# Autodesk Inventor assembly: Trunk
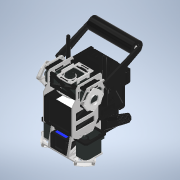
[picture p0: Inventor's stored thumbnail of the model, 180x180]
Saved by Autodesk Inventor 2020.4 (Build 244396000, 396)
## iProperties
Created: 2021-09-10
Part Number: Trunk
Document SubType Name: Assembly
Designer: Masato
Mass: 1534.62 g
Surface Area: 5672.23 cm^2
Volume: 933.606 cm^3
Density: 1.64375 g/cm^3
Author: Masato
## Documents named in this file (25)
- C:\Users\Masato\Documents\Inventor\CIT Brains_Inventor\OpenPlatform_ver3_0\UpperBody\Trunk\Trunk.iam
- C:\Users\Masato\Documents\Inventor\CIT Brains_Inventor\OpenPlatform_ver3_0\UpperBody\Trunk\Trunk_horizontal_frame_01.ipt
- C:\Users\Masato\Documents\Inventor\CIT Brains_Inventor\OpenPlatform_ver3_0\UpperBody\Trunk\Trunk_horizontal_frame_02.ipt
- C:\Users\Masato\Documents\Inventor\CIT Brains_Inventor\OpenPlatform_ver3_0\UpperBody\Trunk\Trunk_horizontal_frame_03.ipt
- C:\Users\Masato\Documents\Inventor\CIT Brains_Inventor\OpenPlatform_ver3_0\UpperBody\Trunk\Trunk_horizontal_frame_04.ipt
- C:\Users\Masato\Documents\Inventor\CIT Brains_Inventor\OpenPlatform_ver3_0\UpperBody\Trunk\Trunk_horizontal_frame_05.ipt
- C:\Users\Masato\Documents\Inventor\CIT Brains_Inventor\OpenPlatform_ver3_0\UpperBody\Trunk\Trunk_vertical_frame_02.ipt
- C:\Users\Masato\Documents\Inventor\CIT Brains_Inventor\OpenPlatform_ver3_0\UpperBody\Trunk\Trunk_vertical_frame_03.ipt
- C:\Users\Masato\Documents\Inventor\CIT Brains_Inventor\OpenPlatform_ver3_0\UpperBody\Trunk\Trunk_vertical_frame_04.ipt
- C:\Users\Masato\Documents\Inventor\CIT Brains_Inventor\OpenPlatform_ver3_0\UpperBody\Trunk\Trunk_vertical_frame_05.ipt
- C:\Users\Masato\Documents\Inventor\CIT Brains_Inventor\OpenPlatform_ver3_0\UpperBody\Trunk\Trunk_vertical_frame_06.ipt
- C:\Users\Masato\Documents\Inventor\CIT Brains_Inventor\OpenPlatform_ver3_0\Ready_Made\B3M11xx.ipt
- C:\Users\Masato\Documents\Inventor\CIT Brains_Inventor\OpenPlatform_ver3_0\Ready_Made\S3-07-3W.ipt
- C:\Users\Masato\Documents\Inventor\CIT Brains_Inventor\OpenPlatform_ver3_0\Ready_Made\ASU-375H.ipt
- C:\Users\Masato\Documents\Inventor\CIT Brains_Inventor\OpenPlatform_ver3_0\UpperBody\Trunk\RearBumper.ipt
- C:\Users\Masato\Documents\Inventor\CIT Brains_Inventor\OpenPlatform_ver3_0\UpperBody\Trunk\RearBumper_MIR.ipt
- C:\Users\Masato\Documents\Inventor\CIT Brains_Inventor\OpenPlatform_ver3_0\Ready_Made\MSU-306-03.ipt
- C:\Users\Masato\Documents\Inventor\CIT Brains_Inventor\OpenPlatform_ver3_0\Ready_Made\SLSBF7-130-M3-N3.ipt
- C:\Users\Masato\Documents\Inventor\CIT Brains_Inventor\OpenPlatform_ver3_0\Ready_Made\B3M10xx.ipt
- C:\Users\Masato\Documents\Inventor\CIT Brains_Inventor\OpenPlatform_ver3_0\Ready_Made\SGB-100.ipt
- C:\Users\Masato\Documents\Inventor\CIT Brains_Inventor\OpenPlatform_ver3_0\UpperBody\Cockpit\Cockpit.iam
- C:\Users\Masato\Documents\Inventor\CIT Brains_Inventor\OpenPlatform_ver3_0\UpperBody\Trunk\Trunk_vertical_frame_04_MIR.ipt
- C:\Users\Masato\Documents\Inventor\CIT Brains_Inventor\OpenPlatform_ver3_0\UpperBody\Trunk\Trunk_vertical_frame_01.ipt
- C:\Users\Masato\Documents\Inventor\CIT Brains_Inventor\OpenPlatform_ver3_0\UpperBody\Trunk\Trunk_vertical_frame_01_MIR.ipt
- C:\Users\Masato\Documents\Inventor\CIT Brains_Inventor\OpenPlatform_ver3_0\下半身\付け根ロール\付け根ロール_サブフレーム_1_3.ipt
## Components (69 placed, 24 different names)
1. Trunk_horizontal_frame_01:1 — メイト:1, フラッシュ:14, 挿入:1, 挿入:2, 挿入:3, 挿入:4, 挿入:5, 挿入:6, 挿入:7, 挿入:8, 挿入:93, 挿入:94, 挿入:95, 挿入:96, 挿入:97, 挿入:98, 挿入:100, 角度:23, 挿入:196, 挿入:197, 挿入:198, 挿入:199, 挿入:211
2. Trunk_horizontal_frame_02:1 — 挿入:9, 挿入:10, 挿入:11, 挿入:12
3. Trunk_horizontal_frame_03:1 — 挿入:172, 挿入:173, 挿入:174, 挿入:175, 挿入:176, 挿入:177, 挿入:178, 挿入:179
4. Trunk_horizontal_frame_03:2 — 挿入:180, 挿入:181, 挿入:182, 挿入:183, 挿入:184, 挿入:185, 挿入:186, 挿入:187
5. Trunk_horizontal_frame_04:1 — 挿入:115, 挿入:116, 挿入:117, 挿入:118, 挿入:172, 挿入:173, 挿入:181, 挿入:182
6. Trunk_horizontal_frame_04:2 — 挿入:154, 挿入:155, 挿入:156, 挿入:157, 挿入:174, 挿入:175, 挿入:185, 挿入:187
7. Trunk_horizontal_frame_05:1 — 挿入:111, 挿入:112, 挿入:126, 挿入:127
8. Trunk_horizontal_frame_05:2 — 挿入:162, 挿入:163, 挿入:164, 挿入:165
9. Trunk_horizontal_frame_05:3 — 挿入:107, 挿入:108, 挿入:138, 挿入:139
10. Trunk_horizontal_frame_05:4 — 挿入:166, 挿入:167, 挿入:168, 挿入:169
11. Trunk_vertical_frame_01:1 — 挿入:196, 挿入:197, 角度:35, 角度:36, 挿入:200, 挿入:201, 挿入:206, 挿入:207
12. Trunk_vertical_frame_01_MIR:1 — 挿入:198, 挿入:199, 角度:37, 角度:38, 挿入:202, 挿入:203, 挿入:204, 挿入:205, メイト:23, メイト:24, メイト:25
13. Trunk_vertical_frame_02:1 — フラッシュ:16, メイト:17, フラッシュ:18, フラッシュ:20, フラッシュ:21, メイト:22
14. Trunk_vertical_frame_02:2 — フラッシュ:16, メイト:17, フラッシュ:18, メイト:19
15. Trunk_vertical_frame_02:3 — フラッシュ:15, メイト:18, フラッシュ:17, フラッシュ:19, フラッシュ:20, フラッシュ:21, メイト:21, メイト:20
16. Trunk_vertical_frame_02:4 — フラッシュ:15, メイト:18, フラッシュ:17, メイト:25
17. Trunk_vertical_frame_03:1 — 挿入:101, 挿入:102, 挿入:103, 挿入:111, 挿入:112, 挿入:115, 挿入:116, 挿入:156, 挿入:157, 挿入:164, 挿入:165, フラッシュ:19, メイト:21, 挿入:208
18. Trunk_vertical_frame_03:2 — 挿入:104, 挿入:105, 挿入:106, 挿入:107, 挿入:108, 挿入:117, 挿入:118, 挿入:154, 挿入:155, 挿入:168, 挿入:169, メイト:22
19. Trunk_vertical_frame_04:1 — 挿入:138, 挿入:139, 挿入:142, 挿入:143, 挿入:144, 挿入:145, 挿入:146, 挿入:147, 挿入:148, 挿入:149, 角度:31, 角度:32, 挿入:150, 挿入:151, 挿入:166, 挿入:167
20. Trunk_vertical_frame_04_MIR:1 — 挿入:124, 挿入:125, 挿入:126, 挿入:127, 挿入:128, 挿入:129, 挿入:132, 挿入:133, 挿入:134, 挿入:135, 挿入:136, 挿入:137, 角度:33, 角度:34, 挿入:152, 挿入:153, 挿入:162, 挿入:163
21. Trunk_vertical_frame_05:1 — 角度:17, 角度:18, 挿入:75, 挿入:76, 角度:21, 挿入:79, メイト:16
22. Trunk_vertical_frame_05:2 — 角度:19, 挿入:77, 挿入:78, 角度:20, 角度:22, 挿入:80
23. Trunk_vertical_frame_06:1 — 挿入:192, 挿入:193, 挿入:194, 挿入:195
24. Trunk_vertical_frame_06:2 — 挿入:188, 挿入:189, 挿入:190, 挿入:191
25. 付け根ロール_サブフレーム_1_3:1 — 挿入:209, 挿入:215, 挿入:216, 挿入:217
26. 付け根ロール_サブフレーム_1_3:2 — 挿入:210, 挿入:212, 挿入:213, 挿入:214
27. 付け根ロール_サブフレーム_1_3:3 — 挿入:221, 挿入:222, 挿入:223, 挿入:224
28. 付け根ロール_サブフレーム_1_3:4 — 挿入:218, 挿入:219, 挿入:220, 挿入:225
29. RearBumper:1 — 挿入:204, 挿入:205
30. RearBumper_MIR:1 — 挿入:206, 挿入:207
31. B3M11xx:1 — 挿入:1, 挿入:2, 挿入:3, 挿入:4, 挿入:11, 挿入:12, 角度:39
32. B3M11xx:2 — 挿入:5, 挿入:6, 挿入:7, 挿入:8, 挿入:9, 挿入:10
33. B3M11xx:3 — 挿入:176, 挿入:177, 挿入:178, 挿入:179, 挿入:180, 挿入:183, 挿入:184, 挿入:186
34. B3M10xx:4 — 挿入:124, 挿入:125, 挿入:128, 挿入:129, 挿入:188, 挿入:189, 挿入:190, 挿入:191
35. B3M10xx:5 — 挿入:142, 挿入:143, 挿入:144, 挿入:145, 挿入:192, 挿入:193, 挿入:194, 挿入:195
36. S3-07-3W:1 — 角度:37, 挿入:202
37. S3-07-3W:2 — 角度:38, 挿入:203
38. S3-07-3W:3 — 角度:36, 挿入:201
39. S3-07-3W:4 — 角度:35, 挿入:200
40. S3-07-3W:5 — 角度:33, 挿入:152
41. S3-07-3W:6 — 角度:34, 挿入:153
42. S3-07-3W:7 — 角度:31, 挿入:150
43. S3-07-3W:8 — 角度:32, 挿入:151
44. ASU-375H:1 — フラッシュ:9, フラッシュ:10, フラッシュ:11, フラッシュ:12, 挿入:101, 挿入:104, メイト:19, メイト:20, メイト:23, メイト:24
45. ASU-375H:2 — フラッシュ:9, フラッシュ:11, 挿入:102, 挿入:105
46. ASU-375H:3 — フラッシュ:10, フラッシュ:12, 挿入:103, 挿入:106
47. MSU-306-03:1 — 角度:12, 挿入:133, 挿入:222
48. MSU-306-03:2 — 角度:10, 角度:11, 角度:12, 挿入:132, 挿入:221
49. MSU-306-03:3 — 角度:11, 挿入:135, 挿入:224
50. MSU-306-03:4 — 角度:10, 挿入:134, 挿入:223
51. MSU-306-03:5 — 角度:17, 挿入:75, 挿入:136
52. MSU-306-03:6 — 角度:18, 挿入:76, 挿入:137
53. MSU-306-03:7 — 角度:14, 角度:15, 角度:16, 挿入:146, 挿入:218
54. MSU-306-03:8 — 角度:14, 挿入:147, 挿入:220
55. MSU-306-03:9 — 角度:15, 挿入:149, 挿入:225
56. MSU-306-03:10 — 角度:16, 挿入:148, 挿入:219
57. MSU-306-03:11 — 角度:19, 挿入:77
58. MSU-306-03:12 — 挿入:78, 角度:20
59. SLSBF7-130-M3-N3:1 — 角度:21, 角度:22, 挿入:79, 挿入:80, メイト:15
60. SGB-100:1 — メイト:15, メイト:16
61. MSU-306-03:13 — 挿入:93, 角度:23, 角度:24, 角度:25, 角度:26, 角度:27, 角度:28, 角度:29, 角度:30, 挿入:217
62. MSU-306-03:14 — 挿入:95, 角度:25, 挿入:209
63. MSU-306-03:15 — 挿入:94, 角度:24, 挿入:216
64. MSU-306-03:16 — 挿入:96, 角度:26, 挿入:215
65. MSU-306-03:17 — 挿入:97, 角度:27, 挿入:210
66. MSU-306-03:18 — 挿入:98, 角度:30, 挿入:214
67. MSU-306-03:19 — 角度:28, 挿入:211, 挿入:212
68. MSU-306-03:20 — 挿入:100, 角度:29, 挿入:213
69. Cockpit:1 [sub-assembly] — 挿入:208, 角度:39
## Relationships (184: Insert 131, Angle 29, Mate 12, Flush 12)
- メイト:1 [Mate]: Trunk_horizontal_frame_01:1
- フラッシュ:14 [Flush]: Trunk_horizontal_frame_01:1
- 挿入:1 [Insert]: Trunk_horizontal_frame_01:1 ↔ B3M11xx:1
- 挿入:2 [Insert]: Trunk_horizontal_frame_01:1 ↔ B3M11xx:1
- 挿入:3 [Insert]: Trunk_horizontal_frame_01:1 ↔ B3M11xx:1
- 挿入:4 [Insert]: Trunk_horizontal_frame_01:1 ↔ B3M11xx:1
- 挿入:5 [Insert]: Trunk_horizontal_frame_01:1 ↔ B3M11xx:2
- 挿入:6 [Insert]: Trunk_horizontal_frame_01:1 ↔ B3M11xx:2
- 挿入:7 [Insert]: Trunk_horizontal_frame_01:1 ↔ B3M11xx:2
- 挿入:8 [Insert]: Trunk_horizontal_frame_01:1 ↔ B3M11xx:2
- 挿入:9 [Insert]: Trunk_horizontal_frame_02:1 ↔ B3M11xx:2
- 挿入:10 [Insert]: Trunk_horizontal_frame_02:1 ↔ B3M11xx:2
- 挿入:11 [Insert]: Trunk_horizontal_frame_02:1 ↔ B3M11xx:1
- 挿入:12 [Insert]: Trunk_horizontal_frame_02:1 ↔ B3M11xx:1
- フラッシュ:9 [Flush]: ASU-375H:1 ↔ ASU-375H:2
- フラッシュ:10 [Flush]: ASU-375H:1 ↔ ASU-375H:3
- フラッシュ:11 [Flush]: ASU-375H:1 ↔ ASU-375H:2
- フラッシュ:12 [Flush]: ASU-375H:1 ↔ ASU-375H:3
- 角度:10 [Angle] (0 deg): MSU-306-03:2 ↔ MSU-306-03:4
- 角度:11 [Angle] (0 deg): MSU-306-03:2 ↔ MSU-306-03:3
- 角度:12 [Angle] (0 deg): MSU-306-03:1 ↔ MSU-306-03:2
- 角度:14 [Angle] (0 deg): MSU-306-03:7 ↔ MSU-306-03:8
- 角度:15 [Angle] (0 deg): MSU-306-03:7 ↔ MSU-306-03:9
- 角度:16 [Angle] (0 deg): MSU-306-03:7 ↔ MSU-306-03:10
- 角度:17 [Angle] (0 deg): Trunk_vertical_frame_05:1 ↔ MSU-306-03:5
- 角度:18 [Angle] (0 deg): Trunk_vertical_frame_05:1 ↔ MSU-306-03:6
- 挿入:75 [Insert]: Trunk_vertical_frame_05:1 ↔ MSU-306-03:5
- 挿入:76 [Insert]: Trunk_vertical_frame_05:1 ↔ MSU-306-03:6
- 角度:19 [Angle] (0 deg): Trunk_vertical_frame_05:2 ↔ MSU-306-03:11
- 挿入:77 [Insert]: Trunk_vertical_frame_05:2 ↔ MSU-306-03:11
- 挿入:78 [Insert]: Trunk_vertical_frame_05:2 ↔ MSU-306-03:12
- 角度:20 [Angle] (0 deg): Trunk_vertical_frame_05:2 ↔ MSU-306-03:12
- 角度:21 [Angle] (0 deg): Trunk_vertical_frame_05:1 ↔ SLSBF7-130-M3-N3:1
- 角度:22 [Angle] (0 deg): Trunk_vertical_frame_05:2 ↔ SLSBF7-130-M3-N3:1
- 挿入:79 [Insert]: Trunk_vertical_frame_05:1 ↔ SLSBF7-130-M3-N3:1
- 挿入:80 [Insert]: Trunk_vertical_frame_05:2 ↔ SLSBF7-130-M3-N3:1
- メイト:15 [Mate]: SLSBF7-130-M3-N3:1 ↔ SGB-100:1
- メイト:16 [Mate] (2.5 mm): Trunk_vertical_frame_05:1 ↔ SGB-100:1
- 挿入:93 [Insert]: Trunk_horizontal_frame_01:1 ↔ MSU-306-03:13
- 挿入:94 [Insert]: Trunk_horizontal_frame_01:1 ↔ MSU-306-03:15
- 挿入:95 [Insert]: Trunk_horizontal_frame_01:1 ↔ MSU-306-03:14
- 挿入:96 [Insert]: Trunk_horizontal_frame_01:1 ↔ MSU-306-03:16
- 挿入:97 [Insert]: Trunk_horizontal_frame_01:1 ↔ MSU-306-03:17
- 挿入:98 [Insert]: Trunk_horizontal_frame_01:1 ↔ MSU-306-03:18
- 挿入:100 [Insert]: Trunk_horizontal_frame_01:1 ↔ MSU-306-03:20
- 角度:23 [Angle] (0 deg): Trunk_horizontal_frame_01:1 ↔ MSU-306-03:13
- 角度:24 [Angle] (0 deg): MSU-306-03:13 ↔ MSU-306-03:15
- 角度:25 [Angle] (0 deg): MSU-306-03:13 ↔ MSU-306-03:14
- 角度:26 [Angle] (0 deg): MSU-306-03:13 ↔ MSU-306-03:16
- 角度:27 [Angle] (0 deg): MSU-306-03:13 ↔ MSU-306-03:17
- 角度:28 [Angle] (0 deg): MSU-306-03:13 ↔ MSU-306-03:19
- 角度:29 [Angle] (0 deg): MSU-306-03:13 ↔ MSU-306-03:20
- 角度:30 [Angle] (0 deg): MSU-306-03:13 ↔ MSU-306-03:18
- 挿入:101 [Insert]: Trunk_vertical_frame_03:1 ↔ ASU-375H:1
- 挿入:102 [Insert]: Trunk_vertical_frame_03:1 ↔ ASU-375H:2
- 挿入:103 [Insert]: Trunk_vertical_frame_03:1 ↔ ASU-375H:3
- 挿入:104 [Insert]: Trunk_vertical_frame_03:2 ↔ ASU-375H:1
- 挿入:105 [Insert]: Trunk_vertical_frame_03:2 ↔ ASU-375H:2
- 挿入:106 [Insert]: Trunk_vertical_frame_03:2 ↔ ASU-375H:3
- 挿入:107 [Insert]: Trunk_horizontal_frame_05:3 ↔ Trunk_vertical_frame_03:2
- 挿入:108 [Insert]: Trunk_horizontal_frame_05:3 ↔ Trunk_vertical_frame_03:2
- 挿入:111 [Insert]: Trunk_horizontal_frame_05:1 ↔ Trunk_vertical_frame_03:1
- 挿入:112 [Insert]: Trunk_horizontal_frame_05:1 ↔ Trunk_vertical_frame_03:1
- 挿入:115 [Insert]: Trunk_horizontal_frame_04:1 ↔ Trunk_vertical_frame_03:1
- 挿入:116 [Insert]: Trunk_horizontal_frame_04:1 ↔ Trunk_vertical_frame_03:1
- 挿入:117 [Insert]: Trunk_horizontal_frame_04:1 ↔ Trunk_vertical_frame_03:2
- 挿入:118 [Insert]: Trunk_horizontal_frame_04:1 ↔ Trunk_vertical_frame_03:2
- 挿入:124 [Insert]: Trunk_vertical_frame_04_MIR:1 ↔ B3M10xx:4
- 挿入:125 [Insert]: Trunk_vertical_frame_04_MIR:1 ↔ B3M10xx:4
- 挿入:126 [Insert]: Trunk_horizontal_frame_05:1 ↔ Trunk_vertical_frame_04_MIR:1
- 挿入:127 [Insert]: Trunk_horizontal_frame_05:1 ↔ Trunk_vertical_frame_04_MIR:1
- 挿入:128 [Insert]: Trunk_vertical_frame_04_MIR:1 ↔ B3M10xx:4
- 挿入:129 [Insert]: Trunk_vertical_frame_04_MIR:1 ↔ B3M10xx:4
- 挿入:132 [Insert]: Trunk_vertical_frame_04_MIR:1 ↔ MSU-306-03:2
- 挿入:133 [Insert]: Trunk_vertical_frame_04_MIR:1 ↔ MSU-306-03:1
- 挿入:134 [Insert]: Trunk_vertical_frame_04_MIR:1 ↔ MSU-306-03:4
- 挿入:135 [Insert]: Trunk_vertical_frame_04_MIR:1 ↔ MSU-306-03:3
- 挿入:136 [Insert]: Trunk_vertical_frame_04_MIR:1 ↔ MSU-306-03:5
- 挿入:137 [Insert]: Trunk_vertical_frame_04_MIR:1 ↔ MSU-306-03:6
- 挿入:138 [Insert]: Trunk_horizontal_frame_05:3 ↔ Trunk_vertical_frame_04:1
- 挿入:139 [Insert]: Trunk_horizontal_frame_05:3 ↔ Trunk_vertical_frame_04:1
- 挿入:142 [Insert]: Trunk_vertical_frame_04:1 ↔ B3M10xx:5
- 挿入:143 [Insert]: Trunk_vertical_frame_04:1 ↔ B3M10xx:5
- 挿入:144 [Insert]: Trunk_vertical_frame_04:1 ↔ B3M10xx:5
- 挿入:145 [Insert]: Trunk_vertical_frame_04:1 ↔ B3M10xx:5
- 挿入:146 [Insert]: Trunk_vertical_frame_04:1 ↔ MSU-306-03:7
- 挿入:147 [Insert]: Trunk_vertical_frame_04:1 ↔ MSU-306-03:8
- 挿入:148 [Insert]: Trunk_vertical_frame_04:1 ↔ MSU-306-03:10
- 挿入:149 [Insert]: Trunk_vertical_frame_04:1 ↔ MSU-306-03:9
- 角度:31 [Angle] (0 deg): Trunk_vertical_frame_04:1 ↔ S3-07-3W:7
- 角度:32 [Angle] (0 deg): Trunk_vertical_frame_04:1 ↔ S3-07-3W:8
- 挿入:150 [Insert]: Trunk_vertical_frame_04:1 ↔ S3-07-3W:7
- 挿入:151 [Insert]: Trunk_vertical_frame_04:1 ↔ S3-07-3W:8
- 角度:33 [Angle] (0 deg): Trunk_vertical_frame_04_MIR:1 ↔ S3-07-3W:5
- 角度:34 [Angle] (0 deg): Trunk_vertical_frame_04_MIR:1 ↔ S3-07-3W:6
- 挿入:152 [Insert]: Trunk_vertical_frame_04_MIR:1 ↔ S3-07-3W:5
- 挿入:153 [Insert]: Trunk_vertical_frame_04_MIR:1 ↔ S3-07-3W:6
- 挿入:154 [Insert]: Trunk_horizontal_frame_04:2 ↔ Trunk_vertical_frame_03:2
- 挿入:155 [Insert]: Trunk_horizontal_frame_04:2 ↔ Trunk_vertical_frame_03:2
- 挿入:156 [Insert]: Trunk_horizontal_frame_04:2 ↔ Trunk_vertical_frame_03:1
- 挿入:157 [Insert]: Trunk_horizontal_frame_04:2 ↔ Trunk_vertical_frame_03:1
- 挿入:162 [Insert]: Trunk_horizontal_frame_05:2 ↔ Trunk_vertical_frame_04_MIR:1
- 挿入:163 [Insert]: Trunk_horizontal_frame_05:2 ↔ Trunk_vertical_frame_04_MIR:1
- 挿入:164 [Insert]: Trunk_horizontal_frame_05:2 ↔ Trunk_vertical_frame_03:1
- 挿入:165 [Insert]: Trunk_horizontal_frame_05:2 ↔ Trunk_vertical_frame_03:1
- 挿入:166 [Insert]: Trunk_horizontal_frame_05:4 ↔ Trunk_vertical_frame_04:1
- 挿入:167 [Insert]: Trunk_horizontal_frame_05:4 ↔ Trunk_vertical_frame_04:1
- 挿入:168 [Insert]: Trunk_horizontal_frame_05:4 ↔ Trunk_vertical_frame_03:2
- 挿入:169 [Insert]: Trunk_horizontal_frame_05:4 ↔ Trunk_vertical_frame_03:2
- 挿入:172 [Insert]: Trunk_horizontal_frame_03:1 ↔ Trunk_horizontal_frame_04:1
- 挿入:173 [Insert]: Trunk_horizontal_frame_03:1 ↔ Trunk_horizontal_frame_04:1
- 挿入:174 [Insert]: Trunk_horizontal_frame_03:1 ↔ Trunk_horizontal_frame_04:2
- 挿入:175 [Insert]: Trunk_horizontal_frame_03:1 ↔ Trunk_horizontal_frame_04:2
- 挿入:176 [Insert]: Trunk_horizontal_frame_03:1 ↔ B3M11xx:3
- 挿入:177 [Insert]: Trunk_horizontal_frame_03:1 ↔ B3M11xx:3
- 挿入:178 [Insert]: Trunk_horizontal_frame_03:1 ↔ B3M11xx:3
- 挿入:179 [Insert]: Trunk_horizontal_frame_03:1 ↔ B3M11xx:3
- 挿入:180 [Insert]: Trunk_horizontal_frame_03:2 ↔ B3M11xx:3
- 挿入:181 [Insert]: Trunk_horizontal_frame_03:2 ↔ Trunk_horizontal_frame_04:1
- 挿入:182 [Insert]: Trunk_horizontal_frame_03:2 ↔ Trunk_horizontal_frame_04:1
- 挿入:183 [Insert]: Trunk_horizontal_frame_03:2 ↔ B3M11xx:3
- 挿入:184 [Insert]: Trunk_horizontal_frame_03:2 ↔ B3M11xx:3
- 挿入:185 [Insert]: Trunk_horizontal_frame_03:2 ↔ Trunk_horizontal_frame_04:2
- 挿入:186 [Insert]: Trunk_horizontal_frame_03:2 ↔ B3M11xx:3
- 挿入:187 [Insert]: Trunk_horizontal_frame_03:2 ↔ Trunk_horizontal_frame_04:2
- 挿入:188 [Insert]: Trunk_vertical_frame_06:2 ↔ B3M10xx:4
- 挿入:189 [Insert]: Trunk_vertical_frame_06:2 ↔ B3M10xx:4
- 挿入:190 [Insert]: Trunk_vertical_frame_06:2 ↔ B3M10xx:4
- 挿入:191 [Insert]: Trunk_vertical_frame_06:2 ↔ B3M10xx:4
- 挿入:192 [Insert]: Trunk_vertical_frame_06:1 ↔ B3M10xx:5
- 挿入:193 [Insert]: Trunk_vertical_frame_06:1 ↔ B3M10xx:5
- 挿入:194 [Insert]: Trunk_vertical_frame_06:1 ↔ B3M10xx:5
- 挿入:195 [Insert]: Trunk_vertical_frame_06:1 ↔ B3M10xx:5
- フラッシュ:15 [Flush]: Trunk_vertical_frame_02:3 ↔ Trunk_vertical_frame_02:4
- フラッシュ:16 [Flush]: Trunk_vertical_frame_02:1 ↔ Trunk_vertical_frame_02:2
- メイト:17 [Mate]: Trunk_vertical_frame_02:1 ↔ Trunk_vertical_frame_02:2
- メイト:18 [Mate]: Trunk_vertical_frame_02:3 ↔ Trunk_vertical_frame_02:4
- フラッシュ:17 [Flush]: Trunk_vertical_frame_02:3 ↔ Trunk_vertical_frame_02:4
- フラッシュ:18 [Flush]: Trunk_vertical_frame_02:1 ↔ Trunk_vertical_frame_02:2
- フラッシュ:19 [Flush]: Trunk_vertical_frame_02:3 ↔ Trunk_vertical_frame_03:1
- フラッシュ:20 [Flush]: Trunk_vertical_frame_02:1 ↔ Trunk_vertical_frame_02:3
- メイト:19 [Mate] (0.01 mm): Trunk_vertical_frame_02:2 ↔ ASU-375H:1
- メイト:20 [Mate] (0.01 mm): Trunk_vertical_frame_02:3 ↔ ASU-375H:1
- フラッシュ:21 [Flush]: Trunk_vertical_frame_02:1 ↔ Trunk_vertical_frame_02:3
- メイト:21 [Mate]: Trunk_vertical_frame_02:3 ↔ Trunk_vertical_frame_03:1
- メイト:22 [Mate]: Trunk_vertical_frame_02:1 ↔ Trunk_vertical_frame_03:2
- 挿入:196 [Insert]: Trunk_horizontal_frame_01:1 ↔ Trunk_vertical_frame_01:1
- 挿入:197 [Insert]: Trunk_horizontal_frame_01:1 ↔ Trunk_vertical_frame_01:1
- 挿入:198 [Insert]: Trunk_horizontal_frame_01:1 ↔ Trunk_vertical_frame_01_MIR:1
- 挿入:199 [Insert]: Trunk_horizontal_frame_01:1 ↔ Trunk_vertical_frame_01_MIR:1
- 角度:35 [Angle] (0 deg): Trunk_vertical_frame_01:1 ↔ S3-07-3W:4
- 角度:36 [Angle] (0 deg): Trunk_vertical_frame_01:1 ↔ S3-07-3W:3
- 挿入:200 [Insert]: Trunk_vertical_frame_01:1 ↔ S3-07-3W:4
- 挿入:201 [Insert]: Trunk_vertical_frame_01:1 ↔ S3-07-3W:3
- 角度:37 [Angle] (0 deg): Trunk_vertical_frame_01_MIR:1 ↔ S3-07-3W:1
- 角度:38 [Angle] (0 deg): Trunk_vertical_frame_01_MIR:1 ↔ S3-07-3W:2
- 挿入:202 [Insert]: Trunk_vertical_frame_01_MIR:1 ↔ S3-07-3W:1
- 挿入:203 [Insert]: Trunk_vertical_frame_01_MIR:1 ↔ S3-07-3W:2
- 挿入:204 [Insert]: Trunk_vertical_frame_01_MIR:1 ↔ RearBumper:1
- 挿入:205 [Insert]: Trunk_vertical_frame_01_MIR:1 ↔ RearBumper:1
- 挿入:206 [Insert]: Trunk_vertical_frame_01:1 ↔ RearBumper_MIR:1
- 挿入:207 [Insert]: Trunk_vertical_frame_01:1 ↔ RearBumper_MIR:1
- メイト:23 [Mate] (0.01 mm): Trunk_vertical_frame_01_MIR:1 ↔ ASU-375H:1
- メイト:24 [Mate] (0.01 mm): Trunk_vertical_frame_01_MIR:1 ↔ ASU-375H:1
- メイト:25 [Mate]: Trunk_vertical_frame_01_MIR:1 ↔ Trunk_vertical_frame_02:4
- 挿入:208 [Insert] (0.25 mm): Trunk_vertical_frame_03:1 ↔ Cockpit:1
- 角度:39 [Angle] (0 deg): B3M11xx:1 ↔ Cockpit:1
- 挿入:209 [Insert]: 付け根ロール_サブフレーム_1_3:1 ↔ MSU-306-03:14
- 挿入:210 [Insert]: 付け根ロール_サブフレーム_1_3:2 ↔ MSU-306-03:17
- 挿入:211 [Insert]: Trunk_horizontal_frame_01:1 ↔ MSU-306-03:19
- 挿入:212 [Insert]: 付け根ロール_サブフレーム_1_3:2 ↔ MSU-306-03:19
- 挿入:213 [Insert]: 付け根ロール_サブフレーム_1_3:2 ↔ MSU-306-03:20
- 挿入:214 [Insert]: 付け根ロール_サブフレーム_1_3:2 ↔ MSU-306-03:18
- 挿入:215 [Insert]: 付け根ロール_サブフレーム_1_3:1 ↔ MSU-306-03:16
- 挿入:216 [Insert]: 付け根ロール_サブフレーム_1_3:1 ↔ MSU-306-03:15
- 挿入:217 [Insert]: 付け根ロール_サブフレーム_1_3:1 ↔ MSU-306-03:13
- 挿入:218 [Insert]: 付け根ロール_サブフレーム_1_3:4 ↔ MSU-306-03:7
- 挿入:219 [Insert]: 付け根ロール_サブフレーム_1_3:4 ↔ MSU-306-03:10
- 挿入:220 [Insert]: 付け根ロール_サブフレーム_1_3:4 ↔ MSU-306-03:8
- 挿入:221 [Insert]: 付け根ロール_サブフレーム_1_3:3 ↔ MSU-306-03:2
- 挿入:222 [Insert]: 付け根ロール_サブフレーム_1_3:3 ↔ MSU-306-03:1
- 挿入:223 [Insert]: 付け根ロール_サブフレーム_1_3:3 ↔ MSU-306-03:4
- 挿入:224 [Insert]: 付け根ロール_サブフレーム_1_3:3 ↔ MSU-306-03:3
- 挿入:225 [Insert]: 付け根ロール_サブフレーム_1_3:4 ↔ MSU-306-03:9
